# Autodesk Inventor assembly: Reaction Ring V0.1
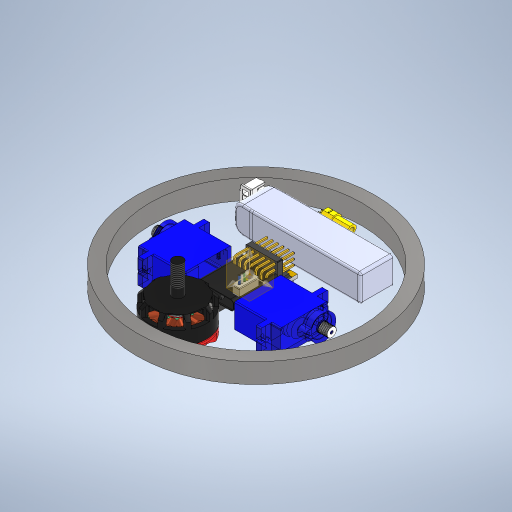
[picture p0: Inventor's stored thumbnail of the model, 512x512]
Saved by Autodesk Inventor 2023.4 (Build 274418000, 418)
## iProperties
Created: 2024-04-30
Part Number: Reaction Ring V0.1
Document SubType Name: Assembly
Designer: Nathan Cai
Mass: 284.695 g
Surface Area: 479.434 cm^2
Volume: 41.0135 cm^3
Density: 6.94148 g/cm^3
Author: Nathan Cai
## Documents named in this file (7)
- E:\Documents\Inventor\Reaction Ring V0.1\Reaction Ring V0.1.iam
- E:\Documents\Inventor\Reaction Ring V0.1\AKK RS2205 2300KV\AKK RS2205 2300KV.iam
- E:\Documents\Inventor\Reaction Ring V0.1\Towerpro Micro Servo 9g\Towerpro Micro Servo 9g.ipt
- E:\Documents\Inventor\Reaction Ring V0.1\Tattu 2S 450mah\Tattu 2S 450mah.iam
- E:\Documents\Inventor\Reaction Ring V0.1\Receiver (FrSky RX6R).ipt
- E:\Documents\Inventor\Reaction Ring V0.1\RDQ ESC32.ipt
- E:\Documents\Inventor\Reaction Ring V0.1\Ring.ipt
## Components (7 placed, 6 different names)
1. AKK RS2205 2300KV:1 [sub-assembly] — Tangent:1
2. Towerpro Micro Servo 9g:1 — Flush:1, Flush:2
3. Towerpro Micro Servo 9g:2 — Flush:1, Flush:2
4. Tattu 2S 450mah:1 [sub-assembly]
5. Receiver (FrSky RX6R):1
6. RDQ ESC32:1
7. Ring:1 — Tangent:1
## Relationships (3: Flush 2, Tangent 1)
- Tangent:1: AKK RS2205 2300KV:1 ↔ Ring:1
- Flush:1: Towerpro Micro Servo 9g:1 ↔ Towerpro Micro Servo 9g:2
- Flush:2: Towerpro Micro Servo 9g:1 ↔ Towerpro Micro Servo 9g:2
